# Autodesk Inventor assembly: 6v dc torque motor
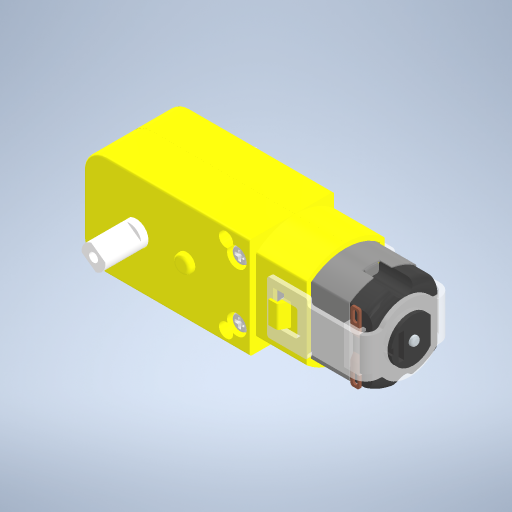
[picture p0: Inventor's stored thumbnail of the model, 512x512]
Saved by Autodesk Inventor 2023.2 (Build 272271000, 271)
## iProperties
Company: Unknown
Created: 2022-10-12
Part Number: 6v dc torque motor
Description: Unknown
Document SubType Name: Assembly
Designer: omrfrkmll
Sending System: DEX
Preprocessor: ST-DEVELOPER v16.7
Title: Moteur
Author: Unknown
## Documents named in this file (11)
- C:\Users\omr_f\Desktop\mechanism design project\6v dc torque motor.iam
- C:\Users\omr_f\Desktop\mechanism design project\Moteur - Enveloppe partie 1 .ipt
- C:\Users\omr_f\Desktop\mechanism design project\Moteur - Engrenage 1.ipt
- C:\Users\omr_f\Desktop\mechanism design project\Moteur - Engrenage 2.ipt
- C:\Users\omr_f\Desktop\mechanism design project\Moteur - Moteur.ipt
- C:\Users\omr_f\Desktop\mechanism design project\Moteur - Axe engrenage.ipt
- C:\Users\omr_f\Desktop\mechanism design project\Moteur - Vis.ipt
- C:\Users\omr_f\Desktop\mechanism design project\Moteur - Enveloppe partie 2.ipt
- C:\Users\omr_f\Desktop\mechanism design project\Moteur - Maintien.ipt
- C:\Users\omr_f\Desktop\mechanism design project\Moteur - Engrenage 3.ipt
- C:\Users\omr_f\Desktop\mechanism design project\Moteur - Engrenage 4.ipt
## Components (11 placed, 10 different names)
1. Moteur - Enveloppe partie 1 — Mate:1, Mate:2
2. Moteur - Engrenage 1 — Mate:1, Mate:2
3. Moteur - Engrenage 2
4. Moteur - Moteur
5. Moteur - Axe engrenage
6. Moteur - Vis
7. Moteur - Vis:1
8. Moteur - Enveloppe partie 2
9. Moteur - Maintien
10. Moteur - Engrenage 3
11. Moteur - Engrenage 4
## Relationships (2: Mate 2)
- Mate:1: Moteur - Enveloppe partie 1 ↔ Moteur - Engrenage 1
- Mate:2: Moteur - Enveloppe partie 1 ↔ Moteur - Engrenage 1
